# Autodesk Inventor assembly: Servo-Arm-38mm-Ball-Joint
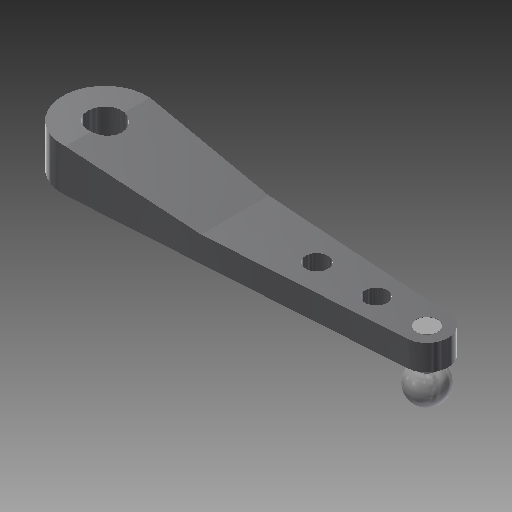
[picture p0: Inventor's stored thumbnail of the model, 512x512]
Saved by Autodesk Inventor 2018.2 (Build 222227000, 227)
## iProperties
Created: 2018-02-18
Part Number: Servo-Arm-38mm-Ball-Joint
Material: Generisch
Document SubType Name: Assembly
Designer: JochenAlt
Author: JochenAlt
## Documents named in this file (3)
- D:\Projects\Donna\CAD\Servo-Arm-38mm-Ball-Joint.iam
- D:\Projects\Donna\CAD\Servo-Arm-38mm.ipt
- D:\Projects\Donna\CAD\Ball-Joint-male.ipt
## Components (2 placed, 2 different names)
1. ServoArm:1 — Passend:1, Passend:2
2. ball joint:1 — Passend:1, Passend:2
## Relationships (2: Mate 2)
- Passend:1 [Mate]: ServoArm:1 ↔ ball joint:1
- Passend:2 [Mate]: ServoArm:1 ↔ ball joint:1
